# Autodesk Inventor assembly: pulley_case
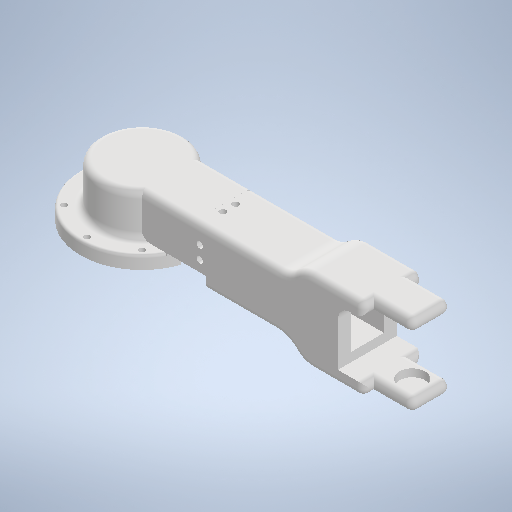
[picture p0: Inventor's stored thumbnail of the model, 512x512]
Saved by Autodesk Inventor 2025 (Build 290162000, 162)
## iProperties
Created: 2025-02-04
Part Number: pulley_case
Document SubType Name: Assembly
Designer: danielrachi
Author: danielrachi
## Documents named in this file (4)
- C:\Users\danielrachi\Documents\pulley_case.iam
- C:\Users\danielrachi\Documents\pulley_case_part_1.ipt
- C:\Users\danielrachi\Documents\pulley_case_part_2.ipt
- C:\Users\danielrachi\Documents\pulley_case_part_3.ipt
## Components (3 placed, 3 different names)
1. pulley_case_part_1:1 — Flush:1, Mate:4, Mate:5
2. pulley_case_part_2:1 — Mate:3, Flush:1, Mate:4, Mate:5
3. pulley_case_part_3:1 — Mate:3
## Relationships (4: Mate 3, Flush 1)
- Mate:3: pulley_case_part_2:1 ↔ pulley_case_part_3:1
- Flush:1: pulley_case_part_1:1 ↔ pulley_case_part_2:1
- Mate:4: pulley_case_part_1:1 ↔ pulley_case_part_2:1
- Mate:5: pulley_case_part_1:1 ↔ pulley_case_part_2:1
